# Autodesk Inventor assembly: ServoMotorAssembly
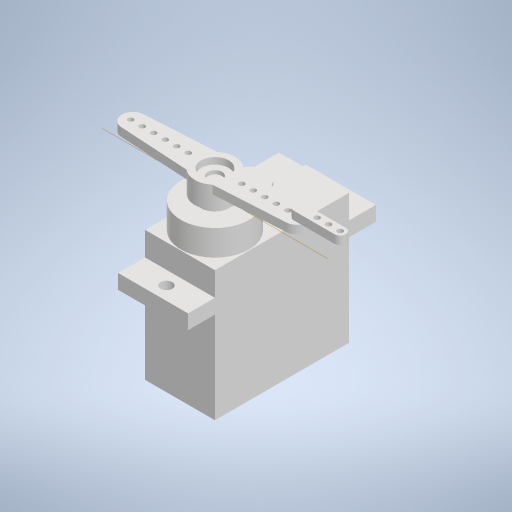
[picture p0: Inventor's stored thumbnail of the model, 512x512]
Saved by Autodesk Inventor 2023 (Build 270158000, 158)
## iProperties
Created: 2023-03-21
Part Number: ServoMotorAssembly
Document SubType Name: Assembly
Designer: 1senadi
Author: 1senadi
## Documents named in this file (4)
- C:\Users\1senadi\Downloads\ServoMotorAssembly.iam
- C:\Users\1senadi\Downloads\Servo Horn.ipt
- C:\Users\1senadi\Downloads\Servo Horn Extension.ipt
- C:\Users\1senadi\Downloads\Servo Motor.ipt
## Components (3 placed, 3 different names)
1. Servo Horn:1 — Insert:1, Insert:2
2. Servo Horn Extension:1 — Insert:1
3. Servo Motor:1 — Insert:2
## Relationships (2: Insert 2)
- Insert:1 (-1.43 mm): Servo Horn:1 ↔ Servo Horn Extension:1
- Insert:2 (-2 mm): Servo Horn:1 ↔ Servo Motor:1
